# Autodesk Inventor assembly: computer assembly
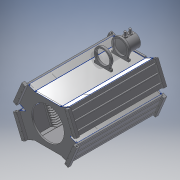
[picture p0: Inventor's stored thumbnail of the model, 180x180]
Saved by Autodesk Inventor 2018 (Build 220112000, 112)
## iProperties
Created: 2018-06-04
Part Number: computer assembly
Document SubType Name: Assembly
Designer: John Viljoen
Author: John Viljoen
## Documents named in this file (12)
- C:\Users\John Viljoen\Documents\Inventor\computer project\computer assembly.iam
- C:\Users\John Viljoen\Documents\Inventor\computer project\baseplate.ipt
- C:\Users\John Viljoen\Documents\Inventor\computer project\coverplate.ipt
- C:\Users\John Viljoen\Documents\Inventor\computer project\topplate.ipt
- C:\Users\John Viljoen\Documents\Inventor\computer project\manifold assembly.iam
- C:\Users\John Viljoen\Documents\Inventor\computer project\manifold assembly_MIR.iam
- C:\Users\John Viljoen\Documents\Inventor\computer project\manifold assembly_MIR1.iam
- C:\Users\John Viljoen\Documents\Inventor\computer project\sideplate part 5.ipt
- C:\Users\John Viljoen\Documents\Inventor\computer project\sideplate part 4.ipt
- C:\Users\John Viljoen\Documents\Inventor\computer project\sideplate part 3.ipt
- C:\Users\John Viljoen\Documents\Inventor\computer project\reservoir pump combo assembly.iam
- C:\Users\John Viljoen\Documents\Inventor\computer project\heat sink.ipt
## Components (19 placed, 11 different names)
1. baseplate:1 — Mate:1, Flush:1, Flush:2, Mate:2, Flush:3, Flush:4, Mate:3, Flush:5, Flush:6, Mate:4, Flush:7, Flush:8, Mate:10, Mate:12, Mate:13, Flush:22, Mate:22, Mate:24, Mate:26, Mate:28
2. coverplate:1 — Mate:1, Flush:1, Flush:2, Flush:18, Mate:14, Mate:21, Flush:23
3. coverplate:2 — Mate:2, Flush:3, Flush:4, Flush:16, Mate:23, Flush:24
4. coverplate:3 — Mate:3, Flush:5, Flush:6, Flush:14, Mate:11, Mate:25, Flush:25
5. coverplate:4 — Mate:4, Flush:7, Flush:8, Mate:5, Flush:9, Flush:10, Flush:11, Flush:12, Mate:27, Flush:26
6. topplate:1 — Mate:5, Flush:9, Flush:10, Mate:6, Mate:7, Flush:13, Mate:8, Flush:15, Mate:9, Flush:17, Flush:19, Mate:15, Flush:20, Mate:17, Flush:21
7. manifold assembly:1 [sub-assembly] — Mate:8, Flush:15, Flush:16
8. manifold assembly:4 [sub-assembly] — Mate:6, Flush:11, Flush:12
9. manifold assembly_MIR:1 [sub-assembly] — Mate:7, Flush:13, Flush:14, Mate:16
10. manifold assembly_MIR1:1 [sub-assembly] — Mate:9, Flush:17, Flush:18, Mate:18
11. sideplate part 5:1 — Mate:10, Mate:11, Mate:12, Mate:19, Mate:20
12. sideplate part 4:1 — Mate:13, Flush:19, Mate:14
13. sideplate part 3:1 — Mate:15, Mate:16, Flush:20
14. sideplate part 3:2 — Mate:17, Mate:18, Flush:21
15. reservoir pump combo assembly:1 [sub-assembly] — Mate:19, Flush:22, Mate:20
16. heat sink:1 — Mate:21, Mate:22, Flush:23
17. heat sink:2 — Mate:23, Mate:24, Flush:24
18. heat sink:3 — Mate:25, Mate:26, Flush:25
19. heat sink:4 — Mate:27, Mate:28, Flush:26
## Relationships (54: Mate 28, Flush 26)
- Mate:1: baseplate:1 ↔ coverplate:1
- Flush:1: baseplate:1 ↔ coverplate:1
- Flush:2: baseplate:1 ↔ coverplate:1
- Mate:2: baseplate:1 ↔ coverplate:2
- Flush:3: baseplate:1 ↔ coverplate:2
- Flush:4: baseplate:1 ↔ coverplate:2
- Mate:3: baseplate:1 ↔ coverplate:3
- Flush:5: baseplate:1 ↔ coverplate:3
- Flush:6: baseplate:1 ↔ coverplate:3
- Mate:4: baseplate:1 ↔ coverplate:4
- Flush:7: baseplate:1 ↔ coverplate:4
- Flush:8: baseplate:1 ↔ coverplate:4
- Mate:5: coverplate:4 ↔ topplate:1
- Flush:9: coverplate:4 ↔ topplate:1
- Flush:10: coverplate:4 ↔ topplate:1
- Mate:6: topplate:1 ↔ manifold assembly:4
- Flush:11: coverplate:4 ↔ manifold assembly:4
- Flush:12 (-9.525 mm): coverplate:4 ↔ manifold assembly:4
- Mate:7: topplate:1 ↔ manifold assembly_MIR:1
- Flush:13: topplate:1 ↔ manifold assembly_MIR:1
- Flush:14 (-9.525 mm): coverplate:3 ↔ manifold assembly_MIR:1
- Mate:8: topplate:1 ↔ manifold assembly:1
- Flush:15: topplate:1 ↔ manifold assembly:1
- Flush:16 (-9.525 mm): coverplate:2 ↔ manifold assembly:1
- Mate:9: topplate:1 ↔ manifold assembly_MIR1:1
- Flush:17: topplate:1 ↔ manifold assembly_MIR1:1
- Flush:18 (-9.525 mm): coverplate:1 ↔ manifold assembly_MIR1:1
- Mate:10: baseplate:1 ↔ sideplate part 5:1
- Mate:11: coverplate:3 ↔ sideplate part 5:1
- Mate:12: baseplate:1 ↔ sideplate part 5:1
- Mate:13: baseplate:1 ↔ sideplate part 4:1
- Flush:19: topplate:1 ↔ sideplate part 4:1
- Mate:14: coverplate:1 ↔ sideplate part 4:1
- Mate:15: topplate:1 ↔ sideplate part 3:1
- Mate:16: manifold assembly_MIR:1 ↔ sideplate part 3:1
- Flush:20: topplate:1 ↔ sideplate part 3:1
- Mate:17: topplate:1 ↔ sideplate part 3:2
- Mate:18: manifold assembly_MIR1:1 ↔ sideplate part 3:2
- Flush:21: topplate:1 ↔ sideplate part 3:2
- Mate:19: sideplate part 5:1 ↔ reservoir pump combo assembly:1
- Flush:22: baseplate:1 ↔ reservoir pump combo assembly:1
- Mate:20: sideplate part 5:1 ↔ reservoir pump combo assembly:1
- Mate:21: coverplate:1 ↔ heat sink:1
- Mate:22: baseplate:1 ↔ heat sink:1
- Flush:23: coverplate:1 ↔ heat sink:1
- Mate:23: coverplate:2 ↔ heat sink:2
- Mate:24: baseplate:1 ↔ heat sink:2
- Flush:24: coverplate:2 ↔ heat sink:2
- Mate:25: coverplate:3 ↔ heat sink:3
- Mate:26: baseplate:1 ↔ heat sink:3
- Flush:25: coverplate:3 ↔ heat sink:3
- Mate:27: coverplate:4 ↔ heat sink:4
- Mate:28: baseplate:1 ↔ heat sink:4
- Flush:26: coverplate:4 ↔ heat sink:4
